# Autodesk Inventor assembly: Drive2
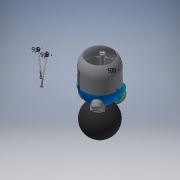
[picture p0: Inventor's stored thumbnail of the model, 180x180]
Saved by Autodesk Inventor 2018.3 (Build 223284000, 284)
## iProperties
Created: 2018-06-30
Part Number: Drive2
Material: Generisch
Document SubType Name: Assembly
Designer: JochenAlt
Author: JochenAlt
## Documents named in this file (5)
- D:\Projects\Ondine\CAD\Drive.iam
- D:\Projects\Ondine\CAD\Sphere.ipt
- D:\Projects\Ondine\CAD\Form.iam
- D:\Projects\Ondine\CAD\DriveChain.iam
- D:\Projects\Ondine\CAD\ControllerPCB.ipt
## Components (4 placed, 4 different names)
1. Sphere:1 — Passend:38, Passend:61
2. Form:1 [sub-assembly] — Passend:59
3. DriveChain:1 [sub-assembly] — Passend:59, Winkel:1, Passend:60, Passend:61
4. ControllerPCB:1 — Winkel:1
## Relationships (5: Mate 4, Angle 1)
- Passend:38 [Mate]: Sphere:1
- Passend:59 [Mate]: Form:1 ↔ DriveChain:1
- Winkel:1 [Angle] (0 deg): DriveChain:1 ↔ ControllerPCB:1
- Passend:60 [Mate]: DriveChain:1
- Passend:61 [Mate] (89 mm): Sphere:1 ↔ DriveChain:1
